# Autodesk Inventor assembly: Engel3mmAssembly
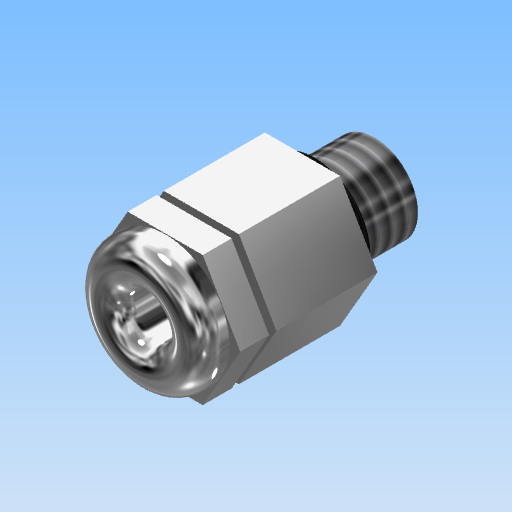
[picture p0: Inventor's stored thumbnail of the model, 512x512]
Saved by Autodesk Inventor 2017 (Build 210142000, 142)
## iProperties
Created: 2016-10-25
Part Number: Engel3mmAssembly
Document SubType Name: Assembly
Designer: techn
Author: techn
## Documents named in this file (4)
- E:\OneDrive\Documents\Other Projects\Submarine\CAD\common\PushRodSeal\Engel3mm\Engel3mmAssembly.iam
- E:\OneDrive\Documents\Other Projects\Submarine\CAD\common\PushRodSeal\Engel3mm\mainBody.ipt
- E:\OneDrive\Documents\Other Projects\Submarine\CAD\common\PushRodSeal\Engel3mm\outerORing.ipt
- E:\OneDrive\Documents\Other Projects\Submarine\CAD\common\PushRodSeal\Engel3mm\sealNut.ipt
## Components (3 placed, 3 different names)
1. mainBody:1 — Mate:1, Mate:2, Rigid:1, Mate:3, Flush:1
2. outerORing:1 — Mate:2, Rigid:1
3. sealNut:1 — Mate:1, Mate:3, Flush:1
## Relationships (5: Mate 3, WeldJoint 1, Flush 1)
- Mate:1: mainBody:1 ↔ sealNut:1
- Mate:2: mainBody:1 ↔ outerORing:1
- Rigid:1 [WeldJoint] (-0.5 mm): mainBody:1 ↔ outerORing:1
- Mate:3: mainBody:1 ↔ sealNut:1
- Flush:1: mainBody:1 ↔ sealNut:1
